# Autodesk Inventor assembly: Knee
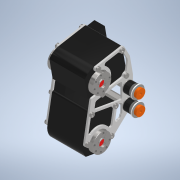
[picture p0: Inventor's stored thumbnail of the model, 180x180]
Saved by Autodesk Inventor 2020 (Build 240168000, 168)
## iProperties
Created: 2021-09-06
Part Number: Knee
Document SubType Name: Assembly
Designer: Masato
Mass: 264.861 g
Surface Area: 473.637 cm^2
Volume: 130.531 cm^3
Density: 2.0291 g/cm^3
Author: Masato
## Documents named in this file (12)
- C:\Users\MasatoKubotera\Documents\Inventor\SUSTAINA-OP\LowerBody\Knee\Knee.iam
- C:\Users\MasatoKubotera\Documents\Inventor\SUSTAINA-OP\LowerBody\Knee\Knee_side_frame.ipt
- C:\Users\MasatoKubotera\Documents\Inventor\SUSTAINA-OP\ReadyMade\Bush\80F-0603.ipt
- C:\Users\MasatoKubotera\Documents\Inventor\SUSTAINA-OP\ReadyMade\Screw\M2_6-15.ipt
- C:\Users\MasatoKubotera\Documents\Inventor\SUSTAINA-OP\ReadyMade\Screw\M2_6-20.ipt
- C:\Users\MasatoKubotera\Documents\Inventor\SUSTAINA-OP\ReadyMade\Spacer\SLSBF6-39.5-M4-N4.ipt
- C:\Users\MasatoKubotera\Documents\Inventor\SUSTAINA-OP\ReadyMade\Washer\UUW-0412-10H.ipt
- C:\Users\MasatoKubotera\Documents\Inventor\SUSTAINA-OP\ReadyMade\Screw\DBTS4-11-8-DHC.ipt
- C:\Users\MasatoKubotera\Documents\Inventor\SUSTAINA-OP\ReadyMade\Washer\TT-0814-10.ipt
- C:\Users\MasatoKubotera\Documents\Inventor\SUSTAINA-OP\ReadyMade\Washer\CCC-0612-65B.ipt
- C:\Users\MasatoKubotera\Documents\Inventor\SUSTAINA-OP\ReadyMade\KONDO\B3M-SC-1170-A_with_ClampHorn_AND_FreeHorn.iam
- C:\Users\MasatoKubotera\Documents\Inventor\SUSTAINA-OP\ReadyMade\Washer\UUW-0614-03H.ipt
## Components (46 placed, 11 different names)
1. B3M-SC-1170-A_with_ClampHorn_AND_FreeHorn:1 [sub-assembly] — 挿入:155, 挿入:156
2. B3M-SC-1170-A_with_ClampHorn_AND_FreeHorn:2 [sub-assembly] — 挿入:157, 挿入:158
3. Knee_side_frame:1 — 挿入:9, 挿入:10, 挿入:12, 挿入:11, 挿入:13, 挿入:14, 挿入:15, 挿入:16, 挿入:33, 挿入:34, 挿入:37, 挿入:38, メイト:1, メイト:2, フラッシュ:1, 角度:1, 挿入:155, 挿入:156, 挿入:157, 挿入:158
4. Knee_side_frame:2 — 挿入:25, 挿入:26, 挿入:27, 挿入:28, 挿入:29, 挿入:30, 挿入:31, 挿入:32, 挿入:35, 挿入:36, 挿入:39, 挿入:40
5. 80F-0603:1 — 挿入:153
6. 80F-0603:2 — 挿入:154
7. 80F-0603:3 — 挿入:151
8. 80F-0603:4 — 挿入:152
9. UUW-0412-10BH:1 — 挿入:37, 挿入:136, 挿入:147
10. UUW-0412-10BH:2 — 挿入:38, 挿入:135, 挿入:148
11. UUW-0412-10BH:3 — 挿入:39, 挿入:137, 挿入:149
12. UUW-0412-10BH:4 — 挿入:40, 挿入:138, 挿入:150
13. SLSBF6-39.5-M4-N4:1 — 挿入:33, 挿入:35, 角度:1, 角度:2
14. SLSBF6-39.5-M4-N4:2 — 挿入:34, 挿入:36, 角度:2
15. DBTS4-11-8:1 — 挿入:138, 挿入:164
16. DBTS4-11-8:2 — 挿入:137, 挿入:163
17. DBTS4-11-8:3 — 挿入:135, 挿入:166
18. DBTS4-11-8:4 — 挿入:136, 挿入:165
19. TT-0814-10:1 — 挿入:161
20. TT-0814-10:2 — 挿入:162
21. TT-0814-10:3 — 挿入:160
22. TT-0814-10:4 — 挿入:159
23. UUW-0614-03H:4 — 挿入:160, 挿入:164
24. UUW-0614-03H:3 — 挿入:159, 挿入:163
25. UUW-0614-03H:2 — 挿入:162, 挿入:166
26. UUW-0614-03H:1 — 挿入:161, 挿入:165
27. CCC-0612-65B:4 — 挿入:150, 挿入:152
28. CCC-0612-65B:3 — 挿入:149, 挿入:151
29. CCC-0612-65B:2 — 挿入:148, 挿入:154
30. CCC-0612-65B:1 — 挿入:147, 挿入:153
31. M2_6-15:1 — 挿入:9
32. M2_6-15:2 — 挿入:10
33. M2_6-15:3 — 挿入:11
34. M2_6-15:4 — 挿入:12
35. M2_6-15:5 — 挿入:13
36. M2_6-15:6 — 挿入:14
37. M2_6-15:7 — 挿入:15
38. M2_6-15:8 — 挿入:16
39. M2_6-20:1 — 挿入:25
40. M2_6-20:2 — 挿入:26
41. M2_6-20:3 — 挿入:27
42. M2_6-20:4 — 挿入:28
43. M2_6-20:5 — 挿入:29
44. M2_6-20:6 — 挿入:30
45. M2_6-20:7 — 挿入:31
46. M2_6-20:8 — 挿入:32
## Relationships (53: Insert 48, Angle 2, Mate 2, Flush 1)
- 挿入:9 [Insert]: Knee_side_frame:1 ↔ M2_6-15:1
- 挿入:10 [Insert]: Knee_side_frame:1 ↔ M2_6-15:2
- 挿入:12 [Insert]: Knee_side_frame:1 ↔ M2_6-15:4
- 挿入:11 [Insert]: Knee_side_frame:1 ↔ M2_6-15:3
- 挿入:13 [Insert]: Knee_side_frame:1 ↔ M2_6-15:5
- 挿入:14 [Insert]: Knee_side_frame:1 ↔ M2_6-15:6
- 挿入:15 [Insert]: Knee_side_frame:1 ↔ M2_6-15:7
- 挿入:16 [Insert]: Knee_side_frame:1 ↔ M2_6-15:8
- 挿入:25 [Insert]: Knee_side_frame:2 ↔ M2_6-20:1
- 挿入:26 [Insert]: Knee_side_frame:2 ↔ M2_6-20:2
- 挿入:27 [Insert]: Knee_side_frame:2 ↔ M2_6-20:3
- 挿入:28 [Insert]: Knee_side_frame:2 ↔ M2_6-20:4
- 挿入:29 [Insert]: Knee_side_frame:2 ↔ M2_6-20:5
- 挿入:30 [Insert]: Knee_side_frame:2 ↔ M2_6-20:6
- 挿入:31 [Insert]: Knee_side_frame:2 ↔ M2_6-20:7
- 挿入:32 [Insert]: Knee_side_frame:2 ↔ M2_6-20:8
- 挿入:33 [Insert]: Knee_side_frame:1 ↔ SLSBF6-39.5-M4-N4:1
- 挿入:34 [Insert]: Knee_side_frame:1 ↔ SLSBF6-39.5-M4-N4:2
- 挿入:35 [Insert]: Knee_side_frame:2 ↔ SLSBF6-39.5-M4-N4:1
- 挿入:36 [Insert]: Knee_side_frame:2 ↔ SLSBF6-39.5-M4-N4:2
- 角度:1 [Angle] (0 deg): Knee_side_frame:1 ↔ SLSBF6-39.5-M4-N4:1
- 角度:2 [Angle] (0 deg): SLSBF6-39.5-M4-N4:1 ↔ SLSBF6-39.5-M4-N4:2
- 挿入:37 [Insert]: Knee_side_frame:1 ↔ UUW-0412-10BH:1
- 挿入:38 [Insert]: Knee_side_frame:1 ↔ UUW-0412-10BH:2
- 挿入:39 [Insert]: Knee_side_frame:2 ↔ UUW-0412-10BH:3
- 挿入:40 [Insert]: Knee_side_frame:2 ↔ UUW-0412-10BH:4
- メイト:1 [Mate]: Knee_side_frame:1
- メイト:2 [Mate] (19.75 mm): Knee_side_frame:1
- フラッシュ:1 [Flush]: Knee_side_frame:1
- 挿入:135 [Insert]: UUW-0412-10BH:2 ↔ DBTS4-11-8:3
- 挿入:136 [Insert]: UUW-0412-10BH:1 ↔ DBTS4-11-8:4
- 挿入:137 [Insert]: UUW-0412-10BH:3 ↔ DBTS4-11-8:2
- 挿入:138 [Insert]: UUW-0412-10BH:4 ↔ DBTS4-11-8:1
- 挿入:147 [Insert]: UUW-0412-10BH:1 ↔ CCC-0612-65B:1
- 挿入:148 [Insert]: UUW-0412-10BH:2 ↔ CCC-0612-65B:2
- 挿入:149 [Insert]: UUW-0412-10BH:3 ↔ CCC-0612-65B:3
- 挿入:150 [Insert]: UUW-0412-10BH:4 ↔ CCC-0612-65B:4
- 挿入:151 [Insert]: 80F-0603:3 ↔ CCC-0612-65B:3
- 挿入:152 [Insert]: 80F-0603:4 ↔ CCC-0612-65B:4
- 挿入:153 [Insert]: 80F-0603:1 ↔ CCC-0612-65B:1
- 挿入:154 [Insert]: 80F-0603:2 ↔ CCC-0612-65B:2
- 挿入:155 [Insert]: B3M-SC-1170-A_with_ClampHorn_AND_FreeHorn:1 ↔ Knee_side_frame:1
- 挿入:156 [Insert]: B3M-SC-1170-A_with_ClampHorn_AND_FreeHorn:1 ↔ Knee_side_frame:1
- 挿入:157 [Insert]: B3M-SC-1170-A_with_ClampHorn_AND_FreeHorn:2 ↔ Knee_side_frame:1
- 挿入:158 [Insert]: B3M-SC-1170-A_with_ClampHorn_AND_FreeHorn:2 ↔ Knee_side_frame:1
- 挿入:159 [Insert]: TT-0814-10:4 ↔ UUW-0614-03H:3
- 挿入:160 [Insert]: TT-0814-10:3 ↔ UUW-0614-03H:4
- 挿入:161 [Insert]: TT-0814-10:1 ↔ UUW-0614-03H:1
- 挿入:162 [Insert]: TT-0814-10:2 ↔ UUW-0614-03H:2
- 挿入:163 [Insert]: DBTS4-11-8:2 ↔ UUW-0614-03H:3
- 挿入:164 [Insert]: DBTS4-11-8:1 ↔ UUW-0614-03H:4
- 挿入:165 [Insert]: DBTS4-11-8:4 ↔ UUW-0614-03H:1
- 挿入:166 [Insert]: DBTS4-11-8:3 ↔ UUW-0614-03H:2
